# Autodesk Inventor assembly: Assembly3
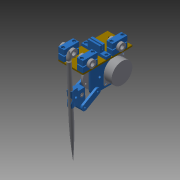
[picture p0: Inventor's stored thumbnail of the model, 180x180]
Saved by Autodesk Inventor 2013 SP2 (Build 170200200, 200)
## iProperties
Created: 2017-01-25
Part Number: Assembly3
Document SubType Name: Assembly
Designer: Herman de Vries
Author: Herman de Vries
## Documents named in this file (7)
- E:\_hdv\Projects\PainterBot\Z Rail assy.iam
- E:\_hdv\Projects\PainterBot\Z Rail.ipt
- E:\_hdv\Projects\PainterBot\brush.ipt
- E:\_hdv\Projects\PainterBot\paint platform assy2.iam
- E:\_hdv\Projects\PainterBot\GT2 grip.ipt
- E:\_hdv\Projects\PainterBot\8mm Rod clamp.ipt
- E:\_hdv\Projects\PainterBot\Linear bearing 8mm.ipt
## Components (13 placed, 6 different names)
1. Z Rail:1 — Mate:15, Mate:18, Flush:10, Flush:11, Mate:23, Mate:24, Mate:25, Flush:13, Flush:14, Flush:16, Flush:17, Flush:18, Flush:20
2. brush:1 — Mate:32, Mate:33
3. paint platform assy2:1 [sub-assembly] — Mate:18, Flush:10, Flush:11, Mate:32, Mate:33
4. GT2 grip:1 — Mate:15, Flush:16, Flush:20
5. 8mm Rod clamp:1 — Mate:23, Insert:3, Mate:31, Flush:17, Flush:19
6. 8mm Rod clamp:2 — Mate:24, Flush:14, Insert:1, Mate:29, Flush:15, Flush:18
7. 8mm Rod clamp:3 — Mate:25, Flush:13, Insert:2, Mate:30, Flush:15, Flush:19
8. Linear bearing 8mm:1 — Insert:1, Mate:28
9. Linear bearing 8mm:2 — Insert:2, Mate:27
10. Linear bearing 8mm:3 — Insert:3, Mate:26
11. 8mm Rod clamp:4 — Mate:26, Mate:31
12. 8mm Rod clamp:5 — Mate:27, Mate:30
13. 8mm Rod clamp:6 — Mate:28, Mate:29
## Relationships (26: Mate 13, Flush 10, Insert 3)
- Mate:15: Z Rail:1 ↔ GT2 grip:1
- Mate:18: Z Rail:1 ↔ paint platform assy2:1
- Flush:10 (15 mm): Z Rail:1 ↔ paint platform assy2:1
- Flush:11 (10 mm): Z Rail:1 ↔ paint platform assy2:1
- Mate:23: Z Rail:1 ↔ 8mm Rod clamp:1
- Mate:24: Z Rail:1 ↔ 8mm Rod clamp:2
- Mate:25: Z Rail:1 ↔ 8mm Rod clamp:3
- Flush:13: Z Rail:1 ↔ 8mm Rod clamp:3
- Flush:14: Z Rail:1 ↔ 8mm Rod clamp:2
- Insert:1 (-5 mm): 8mm Rod clamp:2 ↔ Linear bearing 8mm:1
- Insert:2 (-5 mm): 8mm Rod clamp:3 ↔ Linear bearing 8mm:2
- Insert:3 (-5 mm): 8mm Rod clamp:1 ↔ Linear bearing 8mm:3
- Mate:26: Linear bearing 8mm:3 ↔ 8mm Rod clamp:4
- Mate:27: Linear bearing 8mm:2 ↔ 8mm Rod clamp:5
- Mate:28: Linear bearing 8mm:1 ↔ 8mm Rod clamp:6
- Mate:29: 8mm Rod clamp:2 ↔ 8mm Rod clamp:6
- Mate:30: 8mm Rod clamp:3 ↔ 8mm Rod clamp:5
- Mate:31: 8mm Rod clamp:1 ↔ 8mm Rod clamp:4
- Flush:15: 8mm Rod clamp:2 ↔ 8mm Rod clamp:3
- Flush:16 (47 mm): Z Rail:1 ↔ GT2 grip:1
- Flush:17: Z Rail:1 ↔ 8mm Rod clamp:1
- Flush:18: Z Rail:1 ↔ 8mm Rod clamp:2
- Flush:19 (-60 mm): 8mm Rod clamp:1 ↔ 8mm Rod clamp:3
- Flush:20: Z Rail:1 ↔ GT2 grip:1
- Mate:32: brush:1 ↔ paint platform assy2:1
- Mate:33 (18 mm): brush:1 ↔ paint platform assy2:1
